# Autodesk Inventor assembly: SERVO  KH56KM2U121
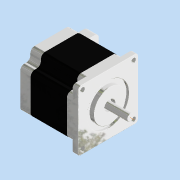
[picture p0: Inventor's stored thumbnail of the model, 180x180]
Saved by Autodesk Inventor 2021 (Build 250183000, 183)
## iProperties
Created: 2021-10-05
Part Number: SERVO  KH56KM2U121
Document SubType Name: Assembly
Designer: 41601100
Author: 41601100
## Documents named in this file (4)
- D:\Ban ve 3d\MAY CNC 300X1200\DONG CO SERVO KH56KM2U121\SERVO  KH56KM2U121.iam
- D:\Ban ve 3d\MAY CNC 300X1200\DONG CO SERVO KH56KM2U121\SERVO  KH56KM2U121 A.ipt
- D:\Ban ve 3d\MAY CNC 300X1200\DONG CO SERVO KH56KM2U121\SERVO  KH56KM2U121 B.ipt
- D:\Ban ve 3d\MAY CNC 300X1200\DONG CO SERVO KH56KM2U121\SERVO  KH56KM2U121 C.ipt
## Components (3 placed, 3 different names)
1. SERVO  KH56KM2U121 A:1 — Mate:1, Mate:2, Mate:3
2. SERVO  KH56KM2U121 B:1 — Mate:1, Mate:2, Mate:3, Mate:4, Mate:5, Mate:6
3. SERVO  KH56KM2U121 C:1 — Mate:4, Mate:5, Mate:6
## Relationships (6: Mate 6)
- Mate:1: SERVO  KH56KM2U121 A:1 ↔ SERVO  KH56KM2U121 B:1
- Mate:2: SERVO  KH56KM2U121 A:1 ↔ SERVO  KH56KM2U121 B:1
- Mate:3: SERVO  KH56KM2U121 A:1 ↔ SERVO  KH56KM2U121 B:1
- Mate:4: SERVO  KH56KM2U121 B:1 ↔ SERVO  KH56KM2U121 C:1
- Mate:5: SERVO  KH56KM2U121 B:1 ↔ SERVO  KH56KM2U121 C:1
- Mate:6: SERVO  KH56KM2U121 B:1 ↔ SERVO  KH56KM2U121 C:1
